# Autodesk Inventor assembly: Final_Assemble
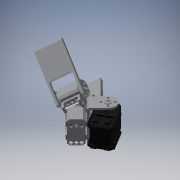
[picture p0: Inventor's stored thumbnail of the model, 180x180]
Saved by Autodesk Inventor 2018 (Build 220112000, 112)
## iProperties
Created: 2018-01-21
Part Number: Final_Assemble
Document SubType Name: Assembly
Designer: wlpeng
Author: wlpeng
## Documents named in this file (12)
- \\engin-labs.m.storage.umich.edu\wlpeng\windat.v2\Desktop\ROB-550\ArmLab_P1\3D_Printing_Files\Final_Assemble.iam
- \\engin-labs.m.storage.umich.edu\wlpeng\windat.v2\Desktop\ROB-550\ArmLab_P1\3D_Printing_Files\Inventor Files\AX12.ipt
- \\engin-labs.m.storage.umich.edu\wlpeng\windat.v2\Desktop\ROB-550\ArmLab_P1\3D_Printing_Files\Inventor Files\AX12_Hub.ipt
- \\engin-labs.m.storage.umich.edu\wlpeng\windat.v2\Desktop\ROB-550\ArmLab_P1\3D_Printing_Files\Inventor Files\AX12_Idler.ipt
- \\engin-labs.m.storage.umich.edu\wlpeng\windat.v2\Desktop\ROB-550\ArmLab_P1\3D_Printing_Files\Inventor Files\OlloHubToBase.ipt
- \\engin-labs.m.storage.umich.edu\wlpeng\windat.v2\Desktop\ROB-550\ArmLab_P1\3D_Printing_Files\Inventor Files\OlloToAX12.ipt
- \\engin-labs.m.storage.umich.edu\wlpeng\windat.v2\Desktop\ROB-550\ArmLab_P1\3D_Printing_Files\Inventor Files\XL320.ipt
- \\engin-labs.m.storage.umich.edu\wlpeng\windat.v2\Desktop\ROB-550\ArmLab_P1\3D_Printing_Files\Inventor Files\XL320_HubToOllo.ipt
- \\engin-labs.m.storage.umich.edu\wlpeng\windat.v2\Desktop\ROB-550\ArmLab_P1\3D_Printing_Files\Inventor Files\XL320_IdlerToOllo.ipt
- \\engin-labs.m.storage.umich.edu\wlpeng\windat.v2\Desktop\ROB-550\ArmLab_P1\3D_Printing_Files\gripper_final.ipt
- \\engin-labs.m.storage.umich.edu\wlpeng\windat.v2\Desktop\ROB-550\ArmLab_P1\3D_Printing_Files\XL320_connecter.ipt
- \\engin-labs.m.storage.umich.edu\wlpeng\windat.v2\Desktop\ROB-550\ArmLab_P1\ROB550 3D CAD Library\Inventor Files\XL320_IdlerToOllo.ipt
## Components (15 placed, 10 different names)
1. AX12:1 — Mate:2, Mate:7
2. AX12_Hub:1 — Mate:2, Mate:3, Mate:4, Mate:7
3. AX12_Idler:1 — Mate:5, Mate:6
4. OlloHubToBase:1 — Mate:13, Mate:14, Mate:15, Mate:16, Mate:17, Mate:18
5. OlloToAX12:1 — Mate:3, Mate:4, Mate:5, Mate:6, Mate:8, Mate:9, Mate:10
6. XL320:1 — Mate:8, Mate:9, Mate:10, Mate:11, Mate:12
7. XL320:2 — Mate:19, Mate:20, Mate:21, Mate:22, Mate:23, Mate:24, Mate:25, Mate:28, Mate:29, Mate:30, Mate:31, Mate:32, Mate:33, Mate:36
8. XL320_HubToOllo:1 — Mate:11, Mate:12, Mate:13, Mate:14, Mate:15
9. XL320_IdlerToOllo:1 — Mate:24, Mate:25
10. gripper_final:1 — Mate:26, Mate:27
11. XL320_connecter:1 — Mate:16, Mate:17, Mate:18, Mate:19, Mate:20, Mate:21
12. XL320_HubToOllo:2 — Mate:22, Mate:23, Mate:26, Mate:27
13. gripper_final:2 — Mate:34, Mate:35, Mate:36
14. XL320_IdlerToOllo:2 — Mate:28, Mate:29, Mate:30
15. XL320_IdlerToOllo:3 — Mate:31, Mate:32, Mate:33, Mate:34, Mate:35
## Relationships (35: Mate 35)
- Mate:2: AX12:1 ↔ AX12_Hub:1
- Mate:3: AX12_Hub:1 ↔ OlloToAX12:1
- Mate:4: AX12_Hub:1 ↔ OlloToAX12:1
- Mate:5: AX12_Idler:1 ↔ OlloToAX12:1
- Mate:6: AX12_Idler:1 ↔ OlloToAX12:1
- Mate:7: AX12:1 ↔ AX12_Hub:1
- Mate:8: OlloToAX12:1 ↔ XL320:1
- Mate:9: OlloToAX12:1 ↔ XL320:1
- Mate:10: OlloToAX12:1 ↔ XL320:1
- Mate:11: XL320:1 ↔ XL320_HubToOllo:1
- Mate:12: XL320:1 ↔ XL320_HubToOllo:1
- Mate:13: OlloHubToBase:1 ↔ XL320_HubToOllo:1
- Mate:14: OlloHubToBase:1 ↔ XL320_HubToOllo:1
- Mate:15: OlloHubToBase:1 ↔ XL320_HubToOllo:1
- Mate:16: OlloHubToBase:1 ↔ XL320_connecter:1
- Mate:17: OlloHubToBase:1 ↔ XL320_connecter:1
- Mate:18: OlloHubToBase:1 ↔ XL320_connecter:1
- Mate:19: XL320:2 ↔ XL320_connecter:1
- Mate:20: XL320:2 ↔ XL320_connecter:1
- Mate:21: XL320:2 ↔ XL320_connecter:1
- Mate:22: XL320:2 ↔ XL320_HubToOllo:2
- Mate:23: XL320:2 ↔ XL320_HubToOllo:2
- Mate:24: XL320:2 ↔ XL320_IdlerToOllo:1
- Mate:25: XL320:2 ↔ XL320_IdlerToOllo:1
- Mate:26: gripper_final:1 ↔ XL320_HubToOllo:2
- Mate:27: gripper_final:1 ↔ XL320_HubToOllo:2
- Mate:28: XL320:2 ↔ XL320_IdlerToOllo:2
- Mate:29: XL320:2 ↔ XL320_IdlerToOllo:2
- Mate:30: XL320:2 ↔ XL320_IdlerToOllo:2
- Mate:31: XL320:2 ↔ XL320_IdlerToOllo:3
- Mate:32: XL320:2 ↔ XL320_IdlerToOllo:3
- Mate:33: XL320:2 ↔ XL320_IdlerToOllo:3
- Mate:34: gripper_final:2 ↔ XL320_IdlerToOllo:3
- Mate:35: gripper_final:2 ↔ XL320_IdlerToOllo:3
- Mate:36: XL320:2 ↔ gripper_final:2
